# Autodesk Inventor assembly: X_GANTRY
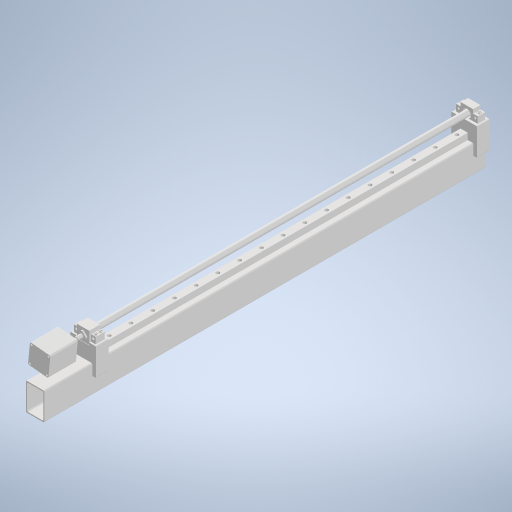
[picture p0: Inventor's stored thumbnail of the model, 512x512]
Saved by Autodesk Inventor 2023 (Build 270158000, 158)
## iProperties
Created: 2022-05-04
Part Number: X_GANTRY
Document SubType Name: Assembly
Designer: plebbb
Author: plebbb
## Documents named in this file (9)
- C:\Users\a laptop\Desktop\CNC_Project\X_GANTRY.iam
- C:\Users\a laptop\Desktop\CNC_Project\2x3_Tube.ipt
- C:\Users\a laptop\Desktop\CNC_Project\HGW20CC_Rail_800mm.ipt
- C:\Users\a laptop\Desktop\CNC_Project\SFU1605_800mm.ipt
- C:\Users\a laptop\Desktop\CNC_Project\BF12.ipt
- C:\Users\a laptop\Desktop\CNC_Project\BK12.ipt
- C:\Users\a laptop\Desktop\CNC_Project\BK12_Spacer.ipt
- C:\Users\a laptop\Desktop\CNC_Project\BF12_Spacer.ipt
- C:\Users\a laptop\Desktop\CNC_Project\Nema23.ipt
## Components (8 placed, 8 different names)
1. 2x3_Tube:1 — Mate:16, Mate:17, Flush:3, Flush:4, Mate:18, Flush:5, Mate:19, Mate:20, Mate:21, Mate:22
2. HGW20CC_Rail_800mm:1 — Flush:4, Mate:18
3. SFU1605_800mm:1
4. BF12:1
5. BK12:1
6. BK12_Spacer:1 — Mate:21, Mate:22
7. BF12_Spacer:1 — Flush:5, Mate:19, Mate:20
8. Nema23:1
## Relationships (22: Mate 18, Flush 4)
- [Mate]: SFU1605_800mm:1 ↔ BK12:1
- [Flush]: SFU1605_800mm:1 ↔ BK12:1
- [Mate]: SFU1605_800mm:1 ↔ BF12:1
- [Mate]: SFU1605_800mm:1 ↔ BF12:1
- [Mate]: BK12:1 ↔ BK12_Spacer:1
- [Mate]: BK12:1 ↔ BK12_Spacer:1
- [Mate]: BK12:1 ↔ BK12_Spacer:1
- [Mate]: BF12:1 ↔ BF12_Spacer:1
- [Mate]: BF12:1 ↔ BF12_Spacer:1
- [Mate]: HGW20CC_Rail_800mm:1 ↔ BF12_Spacer:1
- [Mate]: SFU1605_800mm:1 ↔ Nema23:1
- [Mate]: SFU1605_800mm:1 ↔ Nema23:1
- Mate:16: 2x3_Tube:1
- Mate:17: 2x3_Tube:1
- Flush:3: 2x3_Tube:1
- Flush:4 (15.4 mm): 2x3_Tube:1 ↔ HGW20CC_Rail_800mm:1
- Mate:18: 2x3_Tube:1 ↔ HGW20CC_Rail_800mm:1
- Flush:5: 2x3_Tube:1 ↔ BF12_Spacer:1
- Mate:19: 2x3_Tube:1 ↔ BF12_Spacer:1
- Mate:20: 2x3_Tube:1 ↔ BF12_Spacer:1
- Mate:21: 2x3_Tube:1 ↔ BK12_Spacer:1
- Mate:22: 2x3_Tube:1 ↔ BK12_Spacer:1
